# Autodesk Inventor assembly: RobotAssembly
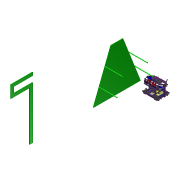
[picture p0: Inventor's stored thumbnail of the model, 180x180]
Saved by Autodesk Inventor 2012 (Build 160160000, 160)
## iProperties
Created: 2013-01-12
Part Number: RobotAssembly
Document SubType Name: Assembly
Designer: JesseK
Mass: 40008.2 g
Surface Area: 561951 cm^2
Volume: 429427 cm^3
Density: 0.0931663 g/cm^3
Author: JesseK
## Documents named in this file (16)
- Z:\UserData\Documents\Inventor\team1885frc\Robot2013\RobotAssembly.iam
- Z:\UserData\Documents\Inventor\team1885frc\Robot2013\DriveTrain\DriveTrainAssembly.iam
- Z:\UserData\Documents\Inventor\team1885frc\Robot2013\Game\floor.ipt
- Z:\UserData\Documents\Inventor\team1885frc\Robot2013\InnerSupportColumn.ipt
- Z:\UserData\Documents\Inventor\team1885frc\Robot2013\MainLiftBlock.ipt
- Z:\UserData\Documents\Inventor\team1885frc\Robot2013\FloorPickup\Frame.iam
- Z:\UserData\Documents\Inventor\team1885frc\Robot2013\CylinderBoundary.ipt
- Z:\UserData\Documents\Inventor\team1885frc\Robot2013\sketches\PyramidMockup.ipt
- Z:\UserData\Documents\Inventor\team1885frc\Pneumatics\0913-DX_13inStrokex10625Bore\0913_DX_R_D_129__F_D_166_1_.iam
- Z:\UserData\Documents\Inventor\team1885frc\Robot2013\sketches\FeederMockup.ipt
- Z:\UserData\Documents\Inventor\team1885frc\Robot2013\DiscTrajectory.ipt
- Z:\UserData\Documents\Inventor\team1885frc\Robot2013\HangHook.ipt
- Z:\UserData\Documents\Inventor\team1885frc\Robot2013\LauncherRearrange\LauncherReassembly.iam
- Z:\UserData\Documents\Inventor\team1885frc\Robot2013\Electronics\ElectronicsAssembly.iam
- Z:\UserData\Documents\Inventor\team1885frc\Hardware\Bolts\Bolt_0.25_20_1.25len_SocketHead.ipt
- Z:\UserData\Documents\Inventor\team1885frc\Hardware\Nuts\LockNut_0.25_20.ipt
## Components (20 placed, 15 different names)
1. DriveTrainAssembly:1 [sub-assembly] — Mate:52, Mate:102, Mate:104, Flush:29, Mate:105, Mate:112, Flush:30, Mate:113
2. InnerSupportColumn:1 — Mate:10, Mate:14, Mate:95, Flush:26, Mate:97
3. InnerSupportColumn:2 — Mate:10, Mate:14, Flush:8, Mate:31, Mate:94, Flush:27, Mate:96, Mate:98, Flush:28, Angle:1
4. MainLiftBlock:1 — Flush:8, Mate:31, Flush:12, Mate:35, Mate:58
5. Frame:1 [sub-assembly] — Mate:112, Flush:30, Mate:113
6. MainLiftBlock:2 — Flush:12, Mate:35, Mate:61
7. floor:1 — Mate:52, Flush:15, Mate:53, Mate:54, Mate:77, Flush:20, Mate:79, Mate:103, Tangent:1
8. PyramidMockup:1 — Flush:15, Mate:53, Mate:54
9. 0913-DX:1 [sub-assembly] — Mate:61
10. 0913-DX:2 [sub-assembly] — Mate:58, Mate:108, Mate:109
11. FeederMockup:1 — Mate:77, Flush:20, Flush:21, Mate:80
12. FeederMockup:2 — Mate:79, Flush:21, Mate:80, Mate:102
13. DiscTrajectory:1 — Mate:99, Mate:101
14. HangHook:1 — Mate:95, Flush:26, Mate:97
15. HangHook:2 — Mate:94, Flush:27, Mate:96
16. LauncherReassembly:1 [sub-assembly] — Mate:98, Flush:28, Angle:1, Mate:99, Mate:101
17. CylinderBoundary:1 — Mate:103, Tangent:1
18. ElectronicsAssembly:1 [sub-assembly] — Mate:104, Flush:29, Mate:105
19. Bolt_0.25_20_1.25len_SocketHead:1 — Mate:108, Mate:109, Mate:111
20. LockNut_0.25_20:1 — Mate:111
## Relationships (40: Mate 28, Flush 10, Angle 1, Tangent 1)
- Mate:10: InnerSupportColumn:1 ↔ InnerSupportColumn:2
- Mate:14: InnerSupportColumn:1 ↔ InnerSupportColumn:2
- Flush:8 (-53.975 mm): InnerSupportColumn:2 ↔ MainLiftBlock:1
- Mate:31: InnerSupportColumn:2 ↔ MainLiftBlock:1
- Flush:12: MainLiftBlock:1 ↔ MainLiftBlock:2
- Mate:35: MainLiftBlock:1 ↔ MainLiftBlock:2
- Mate:52 (25.4 mm): DriveTrainAssembly:1 ↔ floor:1
- Flush:15: floor:1 ↔ PyramidMockup:1
- Mate:53: floor:1 ↔ PyramidMockup:1
- Mate:54: floor:1 ↔ PyramidMockup:1
- Mate:58: MainLiftBlock:1 ↔ 0913-DX:2
- Mate:61: MainLiftBlock:2 ↔ 0913-DX:1
- Mate:77: floor:1 ↔ FeederMockup:1
- Flush:20: floor:1 ↔ FeederMockup:1
- Mate:79: floor:1 ↔ FeederMockup:2
- Flush:21: FeederMockup:1 ↔ FeederMockup:2
- Mate:80 (736.6 mm): FeederMockup:1 ↔ FeederMockup:2
- Mate:94: InnerSupportColumn:2 ↔ HangHook:2
- Mate:95: InnerSupportColumn:1 ↔ HangHook:1
- Flush:26: InnerSupportColumn:1 ↔ HangHook:1
- Flush:27: InnerSupportColumn:2 ↔ HangHook:2
- Mate:96 (-101.6 mm): InnerSupportColumn:2 ↔ HangHook:2
- Mate:97 (-101.6 mm): InnerSupportColumn:1 ↔ HangHook:1
- Mate:98: InnerSupportColumn:2 ↔ LauncherReassembly:1
- Flush:28 (12.7 mm): InnerSupportColumn:2 ↔ LauncherReassembly:1
- Angle:1 (24 deg): InnerSupportColumn:2 ↔ LauncherReassembly:1
- Mate:99: DiscTrajectory:1 ↔ LauncherReassembly:1
- Mate:101: DiscTrajectory:1 ↔ LauncherReassembly:1
- Mate:102: DriveTrainAssembly:1 ↔ FeederMockup:2
- Mate:103: floor:1 ↔ CylinderBoundary:1
- Tangent:1: floor:1 ↔ CylinderBoundary:1
- Mate:104: DriveTrainAssembly:1 ↔ ElectronicsAssembly:1
- Flush:29: DriveTrainAssembly:1 ↔ ElectronicsAssembly:1
- Mate:105: DriveTrainAssembly:1 ↔ ElectronicsAssembly:1
- Mate:108: 0913-DX:2 ↔ Bolt_0.25_20_1.25len_SocketHead:1
- Mate:109: 0913-DX:2 ↔ Bolt_0.25_20_1.25len_SocketHead:1
- Mate:111: Bolt_0.25_20_1.25len_SocketHead:1 ↔ LockNut_0.25_20:1
- Mate:112: DriveTrainAssembly:1 ↔ Frame:1
- Flush:30 (273.05 mm): DriveTrainAssembly:1 ↔ Frame:1
- Mate:113: DriveTrainAssembly:1 ↔ Frame:1
